# Autodesk Inventor assembly: SG90
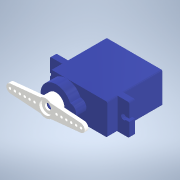
[picture p0: Inventor's stored thumbnail of the model, 180x180]
Saved by Autodesk Inventor 2022.3 (Build 263350000, 350)
## iProperties
Created: 2020-05-29
Part Number: SG90
Document SubType Name: Assembly
Designer: Hagihara Yuya
Mass: 9 g
Surface Area: 32.6562 cm^2
Volume: 7.61914 cm^3
Sending System: Autodesk Translation Framework v8.12.0.6
Preprocessor: ST-DEVELOPER v18
Title: C:/Users/Hagihara Yuya/Documents/Inventor/SirenBuilder/SG90.step
## Documents named in this file (4)
- C:\Users\YusukeKunita\Documents\GrabCAD\Development\BasicParts\ServoMotor\SG90\SG90.iam
- C:\Users\YusukeKunita\Documents\GrabCAD\Development\BasicParts\ServoMotor\SG90\サーボモータ.ipt
- C:\Users\YusukeKunita\Documents\GrabCAD\Development\BasicParts\ServoMotor\SG90\サーボホーン.ipt
- C:\Users\YusukeKunita\Documents\GrabCAD\Development\BasicParts\ServoMotor\SG90\Part6.ipt
## Components (3 placed, 3 different names)
1. サーボモータ:1 — 回転:1, リジッド:1
2. サーボホーン:1 — 回転:1
3. Part6 — リジッド:1
## Relationships (2: RevoluteJoint 1, WeldJoint 1)
- 回転:1 [RevoluteJoint]: サーボモータ:1 ↔ サーボホーン:1
- リジッド:1 [WeldJoint]: サーボモータ:1 ↔ Part6
